# Autodesk Inventor assembly: switch2
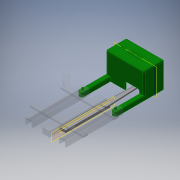
[picture p0: Inventor's stored thumbnail of the model, 180x180]
Saved by Autodesk Inventor 2018 (Build 220112000, 112)
## iProperties
Created: 2017-12-19
Part Number: switch2
Document SubType Name: Assembly
Designer: ragna
Author: ragna
## Documents named in this file (8)
- C:\dev\git\tufftuff\switch2.iam
- C:\dev\git\tufftuff\tracks.ipt
- C:\dev\git\tufftuff\switcher.ipt
- C:\dev\git\tufftuff\servo.ipt
- C:\dev\git\tufftuff\stick.ipt
- C:\dev\git\tufftuff\switchcase2.ipt
- C:\dev\git\tufftuff\jack.ipt
- C:\dev\git\tufftuff\poker2click.ipt
## Components (7 placed, 7 different names)
1. tracks:1 — Flush:1, Mate:1, Mate:2, Flush:4
2. switcher:1 — Flush:1, Mate:1, Mate:2, Flush:5
3. servo:1 — Insert:1, Mate:3
4. stick:1 — Insert:1, Flush:4, Flush:5
5. switchcase2:1 — Mate:3, Insert:2
6. jack:1 — Insert:2
7. poker2click:1
## Relationships (8: Flush 3, Mate 3, Insert 2)
- Flush:1 (-3.5 mm): tracks:1 ↔ switcher:1
- Mate:1: tracks:1 ↔ switcher:1
- Mate:2: tracks:1 ↔ switcher:1
- Insert:1: servo:1 ↔ stick:1
- Flush:4: tracks:1 ↔ stick:1
- Flush:5: switcher:1 ↔ stick:1
- Mate:3: servo:1 ↔ switchcase2:1
- Insert:2: switchcase2:1 ↔ jack:1
